# Autodesk Inventor assembly: Pakiet_blaczek_g
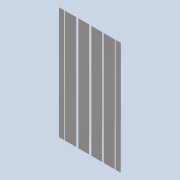
[picture p0: Inventor's stored thumbnail of the model, 180x180]
Saved by Autodesk Inventor 2021.3 (Build 253353000, 353)
## iProperties
Created: 2023-05-23
Part Number: Pakiet_blaczek_g
Document SubType Name: Assembly
Designer: User
Author: User
## Documents named in this file (4)
- E:\Inventor\Projekty\Modele Robotyzacja Procesów\Pakiet_blaczek_g.iam
- E:\Inventor\Projekty\Modele Robotyzacja Procesów\tasiemka_do_zgrzewania_1.ipt
- tasiemka_do_zgrzewania_1.ipt
- E:\Inventor\Projekty\Modele Robotyzacja Procesów\tasiemka_do_zgrzewania_3.ipt
## Components (6 placed, 2 different names)
1. tasiemka_do_zgrzewania_1:1 — Równoległe:8, Równoległe:9, Zestawiające:8
2. tasiemka_do_zgrzewania_1:2 — Równoległe:7, Równoległe:10, Zestawiające:5
3. tasiemka_do_zgrzewania_3:1 — Równoległe:7, Zestawiające:5, Zestawiające:6
4. tasiemka_do_zgrzewania_3:2 — Równoległe:10, Zestawiające:6, Zestawiające:7
5. tasiemka_do_zgrzewania_3:3 — Równoległe:9, Zestawiające:7
6. tasiemka_do_zgrzewania_3:4 — Równoległe:8, Zestawiające:8
## Relationships (8: Flush 4, Mate 4)
- Równoległe:7 [Flush]: tasiemka_do_zgrzewania_1:2 ↔ tasiemka_do_zgrzewania_3:1
- Równoległe:8 [Flush]: tasiemka_do_zgrzewania_1:1 ↔ tasiemka_do_zgrzewania_3:4
- Równoległe:9 [Flush]: tasiemka_do_zgrzewania_1:1 ↔ tasiemka_do_zgrzewania_3:3
- Równoległe:10 [Flush]: tasiemka_do_zgrzewania_1:2 ↔ tasiemka_do_zgrzewania_3:2
- Zestawiające:5 [Mate] (10 mm): tasiemka_do_zgrzewania_1:2 ↔ tasiemka_do_zgrzewania_3:1
- Zestawiające:6 [Mate] (15 mm): tasiemka_do_zgrzewania_3:1 ↔ tasiemka_do_zgrzewania_3:2
- Zestawiające:7 [Mate] (20 mm): tasiemka_do_zgrzewania_3:2 ↔ tasiemka_do_zgrzewania_3:3
- Zestawiające:8 [Mate] (10 mm): tasiemka_do_zgrzewania_1:1 ↔ tasiemka_do_zgrzewania_3:4
